# Autodesk Inventor assembly: Intake motor on xrail left motor front
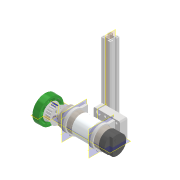
[picture p0: Inventor's stored thumbnail of the model, 180x180]
Saved by Autodesk Inventor 2020 (Build 240168000, 168)
## iProperties
Created: 2020-02-12
Part Number: Intake motor on xrail left motor front
Document SubType Name: Assembly
Designer: ball
Author: ball
## Documents named in this file (3)
- C:\FTC\FTC8863CAD\2019 Robot\Collection\Intake motor on xrail left motor front.iam
- C:\FTC\FTC8863CAD\Actobotics\565 parts\565030.ipt
- C:\FTC\FTC8863CAD\2019 Robot\Collection\neverest 40 + mounts + pulley + compliant wheel + xrail mount.iam
## Components (2 placed, 2 different names)
1. 565030:1 — Mate:1, Mate:2, Flush:1
2. neverest 40 + mounts + pulley + compliant wheel + xrail mount:1 [sub-assembly] — Mate:1, Mate:2, Flush:1
## Relationships (3: Mate 2, Flush 1)
- Mate:1: 565030:1 ↔ neverest 40 + mounts + pulley + compliant wheel + xrail mount:1
- Mate:2: 565030:1 ↔ neverest 40 + mounts + pulley + compliant wheel + xrail mount:1
- Flush:1: 565030:1 ↔ neverest 40 + mounts + pulley + compliant wheel + xrail mount:1
